# Autodesk Inventor assembly: Assy_Motor
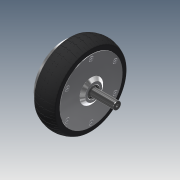
[picture p0: Inventor's stored thumbnail of the model, 180x180]
Saved by Autodesk Inventor 2018 (Build 220112000, 112)
## iProperties
Created: 2017-08-25
Part Number: Assy_Motor
Document SubType Name: Assembly
Designer: Nick Foo
Mass: 3070.86 g
Surface Area: 732.211 cm^2
Volume: 1134.55 cm^3
Density: 2.70669 g/cm^3
Author: Nick Foo
## Documents named in this file (3)
- C:\Users\Nicholas Foo\Google Drive\Hari's Mobility Solution\Design documents\Parts\Assy_Motor.iam
- C:\Users\Nicholas Foo\Google Drive\Hari's Mobility Solution\Design documents\Parts\Motor.ipt
- C:\Users\Nicholas Foo\Documents\Inventor\Content Center Files\R2018\en-US\IFI 513(1)\IFI 513 - M5x0.8 x 10(1) I.ipt
## Components (7 placed, 2 different names)
1. Motor:1
2. Cross Recessed Flat Countersunk Head Machine Screw - Type I - Metric M5x0.8 x 10:1
3. Cross Recessed Flat Countersunk Head Machine Screw - Type I - Metric M5x0.8 x 10:2
4. Cross Recessed Flat Countersunk Head Machine Screw - Type I - Metric M5x0.8 x 10:3
5. Cross Recessed Flat Countersunk Head Machine Screw - Type I - Metric M5x0.8 x 10:4
6. Cross Recessed Flat Countersunk Head Machine Screw - Type I - Metric M5x0.8 x 10:5
7. Cross Recessed Flat Countersunk Head Machine Screw - Type I - Metric M5x0.8 x 10:6
## Relationships (6: Mate 6)
- [Mate]: Motor:1 ↔ Cross Recessed Flat Countersunk Head Machine Screw - Type I - Metric M5x0.8 x 10:1
- [Mate]: Motor:1 ↔ Cross Recessed Flat Countersunk Head Machine Screw - Type I - Metric M5x0.8 x 10:2
- [Mate]: Motor:1 ↔ Cross Recessed Flat Countersunk Head Machine Screw - Type I - Metric M5x0.8 x 10:3
- [Mate]: Motor:1 ↔ Cross Recessed Flat Countersunk Head Machine Screw - Type I - Metric M5x0.8 x 10:4
- [Mate]: Motor:1 ↔ Cross Recessed Flat Countersunk Head Machine Screw - Type I - Metric M5x0.8 x 10:5
- [Mate]: Motor:1 ↔ Cross Recessed Flat Countersunk Head Machine Screw - Type I - Metric M5x0.8 x 10:6
